# Autodesk Inventor assembly: Ground_Antenna230mm
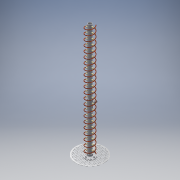
[picture p0: Inventor's stored thumbnail of the model, 180x180]
Saved by Autodesk Inventor 2018 (Build 220112000, 112)
## iProperties
Created: 2018-09-26
Part Number: Ground_Antenna230mm
Document SubType Name: Assembly
Designer: Bradley
Author: Bradley
## Documents named in this file (7)
- C:\Users\Bradley\Documents\GitHub\CougSat1-Hardware\CougSat1-GroundStation\CADModel\Native\Ground_Antenna230mm.iam
- C:\Users\Bradley\Documents\GitHub\CougSat1-Hardware\CougSat1-GroundStation\CADModel\Native\Ground_Antenna230mm_Reflector.ipt
- C:\Users\Bradley\Documents\GitHub\CougSat1-Hardware\CougSat1-GroundStation\CADModel\Native\Ground_Antenna230mm_Helix.ipt
- C:\Users\Bradley\Documents\GitHub\CougSat1-Hardware\CougSat1-GroundStation\CADModel\Native\Ground_Antenna230mm_Support.ipt
- C:\Users\Bradley\Documents\GitHub\CougSat1-Hardware\CougSat1-GroundStation\CADModel\Native\Ground_Antenna230mm_SupportArm.ipt
- C:\Users\Bradley\Documents\GitHub\Resources\ComponentModels\Hardware\Piping_Flange_1.25in.ipt
- C:\Users\Bradley\Documents\GitHub\Resources\ComponentModels\Hardware\Piping_Tee_1.25in.ipt
## Components (49 placed, 6 different names)
1. Ground_Antenna230mm_Reflector:1 — Flush:1, Insert:1, Insert:2
2. Ground_Antenna230mm_Helix:1 — Mate:1, Flush:1, Angle:1, Mate:4, Mate:6
3. Piping_Flange_1.25in:1 — Insert:1, Insert:2, Insert:3
4. Ground_Antenna230mm_Support:1 — Insert:3, Mate:2, Mate:5, Mate:7, Mate:8
5. Piping_Tee_1.25in:1 — Mate:8, Mate:9, Mate:10
6. Ground_Antenna230mm_SupportArm:2 — Mate:5, Mate:6, Flush:2, Mate:7
7. Ground_Antenna230mm_SupportArm:1 — Mate:2, Mate:3, Mate:4
8. Ground_Antenna230mm_SupportArm:3
9. Ground_Antenna230mm_SupportArm:4
10. Ground_Antenna230mm_SupportArm:5
11. Ground_Antenna230mm_SupportArm:6
12. Ground_Antenna230mm_SupportArm:7
13. Ground_Antenna230mm_SupportArm:8
14. Ground_Antenna230mm_SupportArm:9
15. Ground_Antenna230mm_SupportArm:10
16. Ground_Antenna230mm_SupportArm:11
17. Ground_Antenna230mm_SupportArm:12
18. Ground_Antenna230mm_SupportArm:13
19. Ground_Antenna230mm_SupportArm:14
20. Ground_Antenna230mm_SupportArm:15
21. Ground_Antenna230mm_SupportArm:16
22. Ground_Antenna230mm_SupportArm:17
23. Ground_Antenna230mm_SupportArm:18
24. Ground_Antenna230mm_SupportArm:19
25. Ground_Antenna230mm_SupportArm:20
26. Ground_Antenna230mm_SupportArm:21
27. Ground_Antenna230mm_SupportArm:22
28. Ground_Antenna230mm_SupportArm:23
29. Ground_Antenna230mm_SupportArm:24
30. Ground_Antenna230mm_SupportArm:25
31. Ground_Antenna230mm_SupportArm:26
32. Ground_Antenna230mm_SupportArm:27
33. Ground_Antenna230mm_SupportArm:28
34. Ground_Antenna230mm_SupportArm:29
35. Ground_Antenna230mm_SupportArm:30
36. Ground_Antenna230mm_SupportArm:31
37. Ground_Antenna230mm_SupportArm:32
38. Ground_Antenna230mm_SupportArm:33
39. Ground_Antenna230mm_SupportArm:34
40. Ground_Antenna230mm_SupportArm:35
41. Ground_Antenna230mm_SupportArm:36
42. Ground_Antenna230mm_SupportArm:37
43. Ground_Antenna230mm_SupportArm:38
44. Ground_Antenna230mm_SupportArm:39
45. Ground_Antenna230mm_SupportArm:40
46. Ground_Antenna230mm_SupportArm:41
47. Ground_Antenna230mm_SupportArm:42
48. Ground_Antenna230mm_SupportArm:43
49. Ground_Antenna230mm_SupportArm:44
## Component patterns: (22 elements, first: Ground_Antenna230mm_SupportArm:2 + Ground_Antenna230mm_SupportArm:1)
## Relationships (16: Mate 10, Insert 3, Flush 2, Angle 1)
- Mate:1: Ground_Antenna230mm_Helix:1
- Flush:1 (5.375 mm): Ground_Antenna230mm_Reflector:1 ↔ Ground_Antenna230mm_Helix:1
- Insert:1: Ground_Antenna230mm_Reflector:1 ↔ Piping_Flange_1.25in:1
- Insert:2: Ground_Antenna230mm_Reflector:1 ↔ Piping_Flange_1.25in:1
- Insert:3: Piping_Flange_1.25in:1 ↔ Ground_Antenna230mm_Support:1
- Mate:2: Ground_Antenna230mm_Support:1 ↔ Ground_Antenna230mm_SupportArm:1
- Mate:3: Ground_Antenna230mm_SupportArm:1
- Angle:1 (45 deg): Ground_Antenna230mm_Helix:1
- Mate:4 (47.5125 mm): Ground_Antenna230mm_Helix:1 ↔ Ground_Antenna230mm_SupportArm:1
- Mate:5: Ground_Antenna230mm_Support:1 ↔ Ground_Antenna230mm_SupportArm:2
- Mate:6 (20.3625 mm): Ground_Antenna230mm_Helix:1 ↔ Ground_Antenna230mm_SupportArm:2
- Flush:2: Ground_Antenna230mm_SupportArm:2
- Mate:7: Ground_Antenna230mm_Support:1 ↔ Ground_Antenna230mm_SupportArm:2
- Mate:8: Ground_Antenna230mm_Support:1 ↔ Piping_Tee_1.25in:1
- Mate:9 (474 mm): Piping_Tee_1.25in:1
- Mate:10: Piping_Tee_1.25in:1
